# Autodesk Inventor assembly: assembly
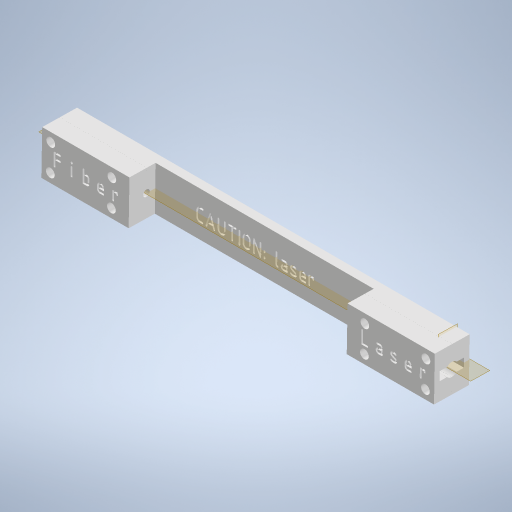
[picture p0: Inventor's stored thumbnail of the model, 512x512]
Saved by Autodesk Inventor 2024 (Build 280153000, 153)
## iProperties
Created: 2023-11-01
Part Number: assembly
Document SubType Name: Assembly
Designer: toybox
Author: toybox
## Documents named in this file (4)
- C:\Users\toybox\Desktop\pw\MAKO\projekt\mako-101_repo\laser_fiber_connector_3D\assembly.iam
- C:\Users\toybox\Desktop\pw\MAKO\projekt\mako-101_repo\laser_fiber_connector_3D\fiber_top.ipt
- C:\Users\toybox\Desktop\pw\MAKO\projekt\mako-101_repo\laser_fiber_connector_3D\lase_top.ipt
- C:\Users\toybox\Desktop\pw\MAKO\projekt\mako-101_repo\laser_fiber_connector_3D\common_bottom.ipt
## Components (3 placed, 3 different names)
1. fiber_top:1 — Mate:3, Mate:4
2. lase_top:1 — Mate:1, Mate:2
3. common_bottom:1 — Mate:1, Mate:2, Mate:3, Mate:4
## Relationships (4: Mate 4)
- Mate:1: lase_top:1 ↔ common_bottom:1
- Mate:2: lase_top:1 ↔ common_bottom:1
- Mate:3: fiber_top:1 ↔ common_bottom:1
- Mate:4: fiber_top:1 ↔ common_bottom:1
